# Autodesk Inventor assembly: Assembly_fridge_new
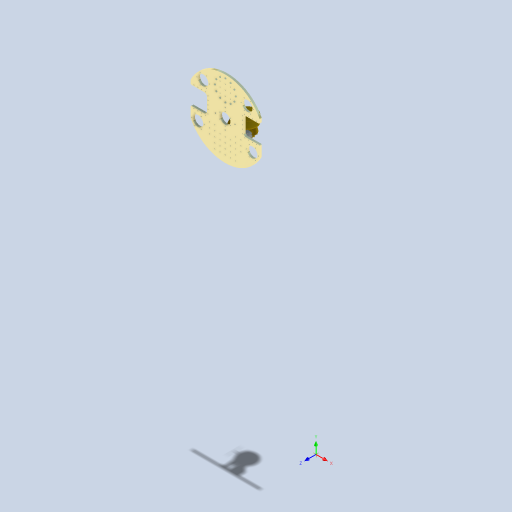
[picture p0: Inventor's stored thumbnail of the model, 512x512]
Saved by Autodesk Inventor 2024 (Build 280153000, 153)
## iProperties
Created: 2023-07-26
Part Number: Assembly_fridge_new
Document SubType Name: Assembly
Designer: gaiadaprato
Author: gaiadaprato
## Documents named in this file (12)
- Z:\People\Gaia\Drawings\Vector_Magnet_Gaia\scripts\GitHub\designs\Inventor\vmag_in_fridge.iam
- Z:\People\Gaia\Drawings\Vector_Magnet_Gaia\scripts\GitHub\designs\Inventor\MXC_Plate_drawing.ipt
- Z:\People\Gaia\Drawings\Vector_Magnet_Gaia\scripts\GitHub\designs\Inventor\attocube_holder.ipt
- Z:\People\Gaia\Drawings\Vector_Magnet_Gaia\scripts\GitHub\designs\Inventor\sample_holder.ipt
- Z:\People\Gaia\Drawings\Vector_Magnet_Gaia\scripts\GitHub\designs\Inventor\Bobbin_x_b.ipt
- Z:\People\Gaia\Drawings\Vector_Magnet_Gaia\scripts\GitHub\designs\Inventor\Bobbin_y_c.ipt
- Z:\People\Gaia\Drawings\Vector_Magnet_Gaia\scripts\GitHub\designs\Inventor\bobbin_support.ipt
- Z:\People\Gaia\Drawings\Vector_Magnet_Gaia\scripts\GitHub\designs\Inventor\Bobbin_z.ipt
- Z:\People\Gaia\Drawings\Vector_Magnet_Gaia\scripts\GitHub\designs\Inventor\ANPx101_RES.ipt
- Z:\People\Gaia\Drawings\Vector_Magnet_Gaia\scripts\GitHub\designs\Inventor\ANPz102_RES.ipt
- Z:\People\Gaia\Drawings\Vector_Magnet_Gaia\scripts\GitHub\designs\Inventor\FiberHolder_v1.ipt
- Z:\People\Gaia\Drawings\Vector_Magnet_Gaia\scripts\GitHub\designs\Inventor\sample.ipt
## Components (12 placed, 11 different names)
1. MXC_Plate_drawing:1 — Mate:1, Mate:2, Symmetry:1, Symmetry:3, Symmetry:5, Mate:16, Angle:2, Mate:17
2. attocube_holder:1 — Mate:1, Symmetry:3, Mate:12, Flush:6, Mate:16
3. sample_holder:1 — Mate:2, Symmetry:1, Mate:4, Mate:5, Mate:6, Mate:7, Mate:13, Flush:7, Mate:15, Symmetry:5, Angle:3, Angle:4, Rotation:2, Rigid:1
4. Bobbin_x_b:1 — Mate:5, Mate:15, Angle:4, Rotation:2, Rigid:1
5. Bobbin_y_c:1 — Mate:4
6. bobbin_support:1 — Mate:3, Symmetry:2, Rotation:1, Angle:1, Mate:6, Mate:7, Angle:3, Mate:18
7. Bobbin_z:1 — Mate:3, Symmetry:2, Rotation:1, Angle:1, Mate:18
8. ANPx101_RES:1 — Mate:9, Flush:1, Flush:2, Mate:10, Flush:3, Flush:4
9. ANPz102_RES:1 — Mate:10, Flush:3, Flush:4, Mate:12, Flush:6
10. ANPx101_RES:2 — Symmetry:4, Mate:9, Flush:1, Flush:2, Mate:11, Flush:5
11. FiberHolder_v1:1 — Symmetry:4, Mate:11, Flush:5
12. sample:1 — Mate:13, Flush:7
## Relationships (35: Mate 16, Flush 7, Symmetry 5, Angle 4, RelateRotation 2, WeldJoint 1)
- Mate:1: MXC_Plate_drawing:1 ↔ attocube_holder:1
- Mate:2: MXC_Plate_drawing:1 ↔ sample_holder:1
- Symmetry:1: MXC_Plate_drawing:1 ↔ sample_holder:1
- Mate:3: bobbin_support:1 ↔ Bobbin_z:1
- Symmetry:2: bobbin_support:1 ↔ Bobbin_z:1
- Rotation:1 [RelateRotation] (1 ul): bobbin_support:1 ↔ Bobbin_z:1
- Angle:1 (90 deg): bobbin_support:1 ↔ Bobbin_z:1
- Mate:4: sample_holder:1 ↔ Bobbin_y_c:1
- Mate:5: sample_holder:1 ↔ Bobbin_x_b:1
- Mate:6: sample_holder:1 ↔ bobbin_support:1
- Mate:7: sample_holder:1 ↔ bobbin_support:1
- Symmetry:3: MXC_Plate_drawing:1 ↔ attocube_holder:1
- Symmetry:4: ANPx101_RES:2 ↔ FiberHolder_v1:1
- Mate:9: ANPx101_RES:1 ↔ ANPx101_RES:2
- Flush:1: ANPx101_RES:1 ↔ ANPx101_RES:2
- Flush:2: ANPx101_RES:1 ↔ ANPx101_RES:2
- Mate:10: ANPx101_RES:1 ↔ ANPz102_RES:1
- Flush:3: ANPx101_RES:1 ↔ ANPz102_RES:1
- Flush:4: ANPx101_RES:1 ↔ ANPz102_RES:1
- Mate:11: ANPx101_RES:2 ↔ FiberHolder_v1:1
- Flush:5: ANPx101_RES:2 ↔ FiberHolder_v1:1
- Mate:12: attocube_holder:1 ↔ ANPz102_RES:1
- Flush:6: attocube_holder:1 ↔ ANPz102_RES:1
- Mate:13: sample_holder:1 ↔ sample:1
- Flush:7: sample_holder:1 ↔ sample:1
- Mate:15: sample_holder:1 ↔ Bobbin_x_b:1
- Symmetry:5: MXC_Plate_drawing:1 ↔ sample_holder:1
- Mate:16: MXC_Plate_drawing:1 ↔ attocube_holder:1
- Angle:2 (180 deg): MXC_Plate_drawing:1
- Mate:17: MXC_Plate_drawing:1
- Angle:3 (0 deg): sample_holder:1 ↔ bobbin_support:1
- Mate:18: bobbin_support:1 ↔ Bobbin_z:1
- Angle:4 (0 deg): sample_holder:1 ↔ Bobbin_x_b:1
- Rotation:2 [RelateRotation] (1 ul): sample_holder:1 ↔ Bobbin_x_b:1
- Rigid:1 [WeldJoint]: sample_holder:1 ↔ Bobbin_x_b:1
